# Autodesk Inventor assembly: 조립품2
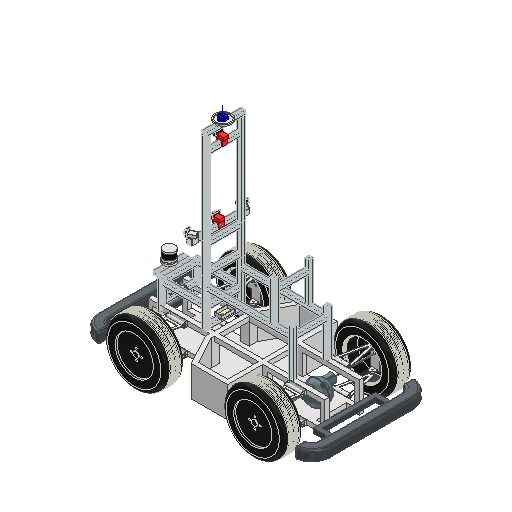
[picture p0: Inventor's stored thumbnail of the model, 512x512]
Saved by Autodesk Inventor 2025.2 (Build 292293000, 293)
## iProperties
Created: 2025-01-26
Part Number: 조립품2
Document SubType Name: Assembly
Designer: jbhma
Author: jbhma
## Documents named in this file (29)
- C:\Users\jbhma\OneDrive\Desktop\2025_ACCA\25_Car\Car1.iam
- C:\Users\jbhma\OneDrive\Desktop\2025_ACCA\2024 ERP42\body.ipt
- C:\Users\jbhma\OneDrive\Desktop\2025_ACCA\2024 ERP42\body_braket.ipt
- C:\Users\jbhma\OneDrive\Desktop\2025_ACCA\2024 ERP42\프로파일\40.5.ipt
- C:\Users\jbhma\OneDrive\Desktop\2025_ACCA\2024 ERP42\프로파일\71.ipt
- C:\Users\jbhma\OneDrive\Desktop\2025_ACCA\2024 ERP42\프로파일\34.ipt
- C:\Users\jbhma\OneDrive\Desktop\2025_ACCA\2024 ERP42\프로파일\26.ipt
- C:\Users\jbhma\OneDrive\Desktop\2025_ACCA\2024 ERP42\프로파일\79.ipt
- C:\Users\jbhma\OneDrive\Desktop\2025_ACCA\2024 ERP42\bumper.ipt
- C:\Users\jbhma\OneDrive\Desktop\2025_ACCA\2024 ERP42\link.ipt
- C:\Users\jbhma\OneDrive\Desktop\2025_ACCA\2024 ERP42\wheel_bolt.ipt
- C:\Users\jbhma\OneDrive\Desktop\2025_ACCA\2024 ERP42\wheel_braket_13.ipt
- C:\Users\jbhma\OneDrive\Desktop\2025_ACCA\2024 ERP42\wheel_braket_24.ipt
- C:\Users\jbhma\OneDrive\Desktop\2025_ACCA\2024 ERP42\wheel.ipt
- C:\Users\jbhma\OneDrive\Desktop\2025_ACCA\2024 ERP42\base_link.ipt
- base_link.ipt
- C:\Users\jbhma\OneDrive\Desktop\2025_ACCA\2024 ERP42\프로파일\50.ipt
- C:\Users\jbhma\OneDrive\Desktop\2025_ACCA\2024 ERP42\camera_case_front.ipt
- C:\Users\jbhma\OneDrive\Desktop\2025_ACCA\2024 ERP42\camera_case_left.ipt
- C:\Users\jbhma\OneDrive\Desktop\2025_ACCA\2024 ERP42\camera_case_right.ipt
- C:\Users\jbhma\OneDrive\Desktop\2025_ACCA\2024 ERP42\camera.ipt
- C:\Users\jbhma\OneDrive\Desktop\2025_ACCA\2024 ERP42\lidar_case.ipt
- C:\Users\jbhma\OneDrive\Desktop\2025_ACCA\2024 ERP42\imu_case_new.ipt
- C:\Users\jbhma\OneDrive\Desktop\2025_ACCA\2024 ERP42\gps_case.ipt
- C:\Users\jbhma\OneDrive\Desktop\2025_ACCA\2024 ERP42\UBLOX_ANN-MB-00_GNSS_ANTENNA.ipt
- C:\Users\jbhma\OneDrive\Desktop\2025_ACCA\2024 ERP42\lidar.ipt
- C:\Users\jbhma\OneDrive\Desktop\2025_ACCA\2024 ERP42\MTi 600-series STEP files\MTi-600 DEV assembly.iam
- C:\Users\jbhma\OneDrive\Desktop\2025_ACCA\2024 ERP42\MTi 600-series STEP files\MTi 1-s DK GNSS.iam
- C:\Users\jbhma\OneDrive\Desktop\2025_ACCA\2024 ERP42\gps_case_2.ipt
## Components (81 placed, 27 different names)
1. body:1 — 메이트:113, 메이트:114, 메이트:115, 메이트:116, 메이트:117, 메이트:118, 메이트:119, 메이트:120, 메이트:124, 메이트:125, 메이트:126, 메이트:127, 메이트:128, 메이트:131, 메이트:137, 메이트:139, 메이트:191, 메이트:192, 메이트:193, 메이트:194, 메이트:195, 메이트:196, 메이트:197, 메이트:198, 메이트:199, 메이트:200, 메이트:201, 메이트:202, 메이트:203, 메이트:204, 메이트:205, 메이트:206
2. body_braket:9 — 메이트:113, 메이트:114, 메이트:212
3. body_braket:10 — 메이트:115, 메이트:116, 메이트:211
4. body_braket:11 — 메이트:117, 메이트:118, 메이트:213
5. body_braket:12 — 메이트:119, 메이트:120, 메이트:214
6. body_braket:13 — 메이트:191, 메이트:195, 메이트:199, 메이트:215
7. body_braket:14 — 메이트:193, 메이트:197, 메이트:202, 메이트:217
8. body_braket:15 — 메이트:194, 메이트:198, 메이트:201, 메이트:218
9. body_braket:16 — 메이트:192, 메이트:196, 메이트:200, 메이트:216
10. bumper:1 — 메이트:203, 메이트:204
11. bumper:2 — 메이트:205, 메이트:206
12. 40.5:12 — 메이트:126, 메이트:127, 메이트:130, 메이트:257
13. 40.5:13 — 메이트:124, 메이트:125, 메이트:129
14. 71:1 — 메이트:128, 메이트:129, 메이트:132, 메이트:133, 메이트:138
15. 71:2 — 메이트:130, 메이트:131, 메이트:134, 메이트:135, 메이트:136, 메이트:256
16. 34:1 — 메이트:134, 메이트:135, 메이트:189
17. 34:2 — 메이트:132, 메이트:133, 메이트:190
18. 40.5:15 — 메이트:136, 메이트:137, 메이트:143, 메이트:144, 메이트:145, 메이트:293
19. 40.5:16 — 메이트:138, 메이트:139, 메이트:140, 메이트:141, 메이트:142, 메이트:168, 메이트:180, 메이트:287, 메이트:288
20. 26:1 — 메이트:140, 메이트:141, 메이트:142, 메이트:149, 메이트:150, 메이트:175, 메이트:176, 메이트:178
21. 26:2 — 메이트:143, 메이트:144, 메이트:145, 메이트:151, 메이트:152, 메이트:177
22. 79:1 — 메이트:151, 메이트:152, 메이트:261
23. 79:2 — 메이트:149, 메이트:150, 메이트:153, 메이트:154, 메이트:262, 각도:3
24. 34:3 — 메이트:153, 메이트:154, 메이트:259
25. 34:6 — 메이트:168, 메이트:172, 각도:1, 메이트:179
26. 34:7 — 메이트:296
27. 26:3 — 메이트:172, 각도:1, 메이트:295, 메이트:297
28. 26:5 — 메이트:175, 메이트:176
29. 26:6 — 메이트:177, 메이트:178, 메이트:301
30. 26:7 — 메이트:179, 메이트:180
31. 26:8 — 메이트:258, 메이트:261, 메이트:262
32. 26:10 — 메이트:189, 메이트:190
33. link:5 — 메이트:211, 메이트:226
34. link:6 — 메이트:212, 메이트:224
35. link:7 — 메이트:214, 메이트:227
36. link:8 — 메이트:213, 메이트:225
37. link:12 — 메이트:215, 메이트:219
38. link:13 — 메이트:217, 메이트:223
39. link:14 — 메이트:216, 메이트:220
40. link:15 — 메이트:218, 메이트:222
41. wheel_bolt:1 — 메이트:219, 메이트:221
42. wheel_braket_13:1 — 메이트:221, 메이트:236, 메이트:237
43. wheel_braket_24:1 — 메이트:229, 메이트:235, 메이트:238
44. wheel_bolt:2 — 메이트:220
45. wheel_bolt:3 — 메이트:222, 메이트:230
46. wheel_bolt:4 — 메이트:223
47. wheel_bolt:5 — 메이트:224, 메이트:228
48. wheel_bolt:6 — 메이트:225, 메이트:229
49. wheel_bolt:7 — 메이트:226
50. wheel_bolt:8 — 메이트:227
51. wheel_braket_13:2 — 메이트:228, 메이트:232
52. wheel:1 — 메이트:232
53. wheel:2 — 메이트:238
54. wheel_braket_24:2 — 메이트:230, 메이트:234
55. wheel:3 — 메이트:237
56. wheel:4 — 메이트:234
57. base_link:1 — 메이트:235, 메이트:236
58. 26:12 — 메이트:256, 메이트:257
59. gps_case:1 — 메이트:259, 각도:3
60. camera_case_front:2 — 메이트:258, 메이트:278
61. UBLOX_ANN-MB-00_GNSS_ANTENNA:1
62. camera:4 — 메이트:278
63. 26:13 — 메이트:290
64. gps_case_2:1 — 메이트:293, 메이트:294, 강체:1
65. MTi 1-s DK GNSS:1 [sub-assembly] — 강체:1
66. 26:14 — 메이트:287, 메이트:288, 메이트:294
67. MTi-600 DEV assembly:1 [sub-assembly] — 메이트:291, 메이트:292
68. imu_case_new:1 — 메이트:290, 메이트:291, 메이트:292
69. 26:15 — 메이트:295, 메이트:298
70. 26:16 — 메이트:296
71. 26:17 — 메이트:297, 메이트:298, 메이트:299, 메이트:300
72. 26:18 — 메이트:299, 메이트:300, 강체:2
73. lidar_case:1 — 강체:2, 회전:1
74. lidar:1 — 회전:1
75. camera:5 — 메이트:306
76. 50:1 — 메이트:301, 메이트:302, 메이트:303, 메이트:304, 메이트:305
77. camera_case_left:1 — 메이트:302, 메이트:306
78. camera_case_front:3 — 메이트:305, 메이트:307
79. camera:6 — 메이트:307
80. camera:7 — 메이트:308
81. camera_case_right:1 — 메이트:303, 메이트:304, 메이트:308
## Relationships (121: Mate 116, Angle 2, WeldJoint 2, RevoluteJoint 1)
- 메이트:113 [Mate] (195 mm): body:1 ↔ body_braket:9
- 메이트:114 [Mate]: body:1 ↔ body_braket:9
- 메이트:115 [Mate] (195 mm): body:1 ↔ body_braket:10
- 메이트:116 [Mate]: body:1 ↔ body_braket:10
- 메이트:117 [Mate] (155 mm): body:1 ↔ body_braket:11
- 메이트:118 [Mate]: body:1 ↔ body_braket:11
- 메이트:119 [Mate] (155 mm): body:1 ↔ body_braket:12
- 메이트:120 [Mate]: body:1 ↔ body_braket:12
- 메이트:124 [Mate]: body:1 ↔ 40.5:13
- 메이트:125 [Mate] (275 mm): body:1 ↔ 40.5:13
- 메이트:126 [Mate]: body:1 ↔ 40.5:12
- 메이트:127 [Mate] (275 mm): body:1 ↔ 40.5:12
- 메이트:128 [Mate] (300 mm): body:1 ↔ 71:1
- 메이트:129 [Mate]: 40.5:13 ↔ 71:1
- 메이트:130 [Mate]: 40.5:12 ↔ 71:2
- 메이트:131 [Mate] (300 mm): body:1 ↔ 71:2
- 메이트:132 [Mate]: 71:1 ↔ 34:2
- 메이트:133 [Mate] (120 mm): 71:1 ↔ 34:2
- 메이트:134 [Mate]: 71:2 ↔ 34:1
- 메이트:135 [Mate] (120 mm): 71:2 ↔ 34:1
- 메이트:136 [Mate]: 71:2 ↔ 40.5:15
- 메이트:137 [Mate]: body:1 ↔ 40.5:15
- 메이트:138 [Mate]: 71:1 ↔ 40.5:16
- 메이트:139 [Mate]: body:1 ↔ 40.5:16
- 메이트:140 [Mate]: 40.5:16 ↔ 26:1
- 메이트:141 [Mate]: 40.5:16 ↔ 26:1
- 메이트:142 [Mate]: 40.5:16 ↔ 26:1
- 메이트:143 [Mate]: 40.5:15 ↔ 26:2
- 메이트:144 [Mate]: 40.5:15 ↔ 26:2
- 메이트:145 [Mate]: 40.5:15 ↔ 26:2
- 메이트:149 [Mate]: 26:1 ↔ 79:2
- 메이트:150 [Mate]: 26:1 ↔ 79:2
- 메이트:151 [Mate]: 26:2 ↔ 79:1
- 메이트:152 [Mate]: 26:2 ↔ 79:1
- 메이트:153 [Mate]: 79:2 ↔ 34:3
- 메이트:154 [Mate]: 79:2 ↔ 34:3
- 메이트:168 [Mate]: 40.5:16 ↔ 34:6
- 메이트:172 [Mate]: 34:6 ↔ 26:3
- 각도:1 [Angle] (90 deg): 34:6 ↔ 26:3
- 메이트:175 [Mate]: 26:1 ↔ 26:5
- 메이트:176 [Mate]: 26:1 ↔ 26:5
- 메이트:177 [Mate]: 26:2 ↔ 26:6
- 메이트:178 [Mate]: 26:1 ↔ 26:6
- 메이트:179 [Mate]: 34:6 ↔ 26:7
- 메이트:180 [Mate]: 40.5:16 ↔ 26:7
- 메이트:189 [Mate]: 34:1 ↔ 26:10
- 메이트:190 [Mate]: 34:2 ↔ 26:10
- 메이트:191 [Mate]: body:1 ↔ body_braket:13
- 메이트:192 [Mate]: body:1 ↔ body_braket:16
- 메이트:193 [Mate]: body:1 ↔ body_braket:14
- 메이트:194 [Mate]: body:1 ↔ body_braket:15
- 메이트:195 [Mate]: body:1 ↔ body_braket:13
- 메이트:196 [Mate]: body:1 ↔ body_braket:16
- 메이트:197 [Mate]: body:1 ↔ body_braket:14
- 메이트:198 [Mate]: body:1 ↔ body_braket:15
- 메이트:199 [Mate] (155 mm): body:1 ↔ body_braket:13
- 메이트:200 [Mate] (155 mm): body:1 ↔ body_braket:16
- 메이트:201 [Mate] (195 mm): body:1 ↔ body_braket:15
- 메이트:202 [Mate] (195 mm): body:1 ↔ body_braket:14
- 메이트:203 [Mate]: body:1 ↔ bumper:1
- 메이트:204 [Mate] (100 mm): body:1 ↔ bumper:1
- 메이트:205 [Mate]: body:1 ↔ bumper:2
- 메이트:206 [Mate] (100 mm): body:1 ↔ bumper:2
- 메이트:211 [Mate]: body_braket:10 ↔ link:5
- 메이트:212 [Mate]: body_braket:9 ↔ link:6
- 메이트:213 [Mate]: body_braket:11 ↔ link:8
- 메이트:214 [Mate]: body_braket:12 ↔ link:7
- 메이트:215 [Mate]: body_braket:13 ↔ link:12
- 메이트:216 [Mate]: body_braket:16 ↔ link:14
- 메이트:217 [Mate]: body_braket:14 ↔ link:13
- 메이트:218 [Mate]: body_braket:15 ↔ link:15
- 메이트:219 [Mate]: link:12 ↔ wheel_bolt:1
- 메이트:220 [Mate]: link:14 ↔ wheel_bolt:2
- 메이트:221 [Mate]: wheel_bolt:1 ↔ wheel_braket_13:1
- 메이트:222 [Mate]: link:15 ↔ wheel_bolt:3
- 메이트:223 [Mate]: link:13 ↔ wheel_bolt:4
- 메이트:224 [Mate]: link:6 ↔ wheel_bolt:5
- 메이트:225 [Mate]: link:8 ↔ wheel_bolt:6
- 메이트:226 [Mate]: link:5 ↔ wheel_bolt:7
- 메이트:227 [Mate]: link:7 ↔ wheel_bolt:8
- 메이트:228 [Mate]: wheel_bolt:5 ↔ wheel_braket_13:2
- 메이트:229 [Mate]: wheel_braket_24:1 ↔ wheel_bolt:6
- 메이트:230 [Mate]: wheel_bolt:3 ↔ wheel_braket_24:2
- 메이트:232 [Mate]: wheel_braket_13:2 ↔ wheel:1
- 메이트:234 [Mate]: wheel_braket_24:2 ↔ wheel:4
- 메이트:235 [Mate]: wheel_braket_24:1 ↔ base_link:1
- 메이트:236 [Mate]: wheel_braket_13:1 ↔ base_link:1
- 메이트:237 [Mate]: wheel_braket_13:1 ↔ wheel:3
- 메이트:238 [Mate]: wheel_braket_24:1 ↔ wheel:2
- 메이트:256 [Mate]: 71:2 ↔ 26:12
- 메이트:257 [Mate]: 40.5:12 ↔ 26:12
- 메이트:258 [Mate]: 26:8 ↔ camera_case_front:2
- 메이트:259 [Mate]: 34:3 ↔ gps_case:1
- 메이트:261 [Mate]: 79:1 ↔ 26:8
- 메이트:262 [Mate]: 79:2 ↔ 26:8
- 각도:3 [Angle] (90 deg): 79:2 ↔ gps_case:1
- 메이트:278 [Mate]: camera_case_front:2 ↔ camera:4
- 메이트:287 [Mate]: 40.5:16 ↔ 26:14
- 메이트:288 [Mate]: 40.5:16 ↔ 26:14
- 메이트:290 [Mate]: 26:13 ↔ imu_case_new:1
- 메이트:291 [Mate]: MTi-600 DEV assembly:1 ↔ imu_case_new:1
- 메이트:292 [Mate]: MTi-600 DEV assembly:1 ↔ imu_case_new:1
- 메이트:293 [Mate] (72.5 mm): 40.5:15 ↔ gps_case_2:1
- 메이트:294 [Mate]: gps_case_2:1 ↔ 26:14
- 강체:1 [WeldJoint]: gps_case_2:1 ↔ MTi 1-s DK GNSS:1
- 메이트:295 [Mate]: 26:3 ↔ 26:15
- 메이트:296 [Mate]: 34:7 ↔ 26:16
- 메이트:297 [Mate]: 26:3 ↔ 26:17
- 메이트:298 [Mate]: 26:15 ↔ 26:17
- 메이트:299 [Mate]: 26:17 ↔ 26:18
- 메이트:300 [Mate]: 26:17 ↔ 26:18
- 강체:2 [WeldJoint]: 26:18 ↔ lidar_case:1
- 회전:1 [RevoluteJoint]: lidar_case:1 ↔ lidar:1
- 메이트:301 [Mate]: 26:6 ↔ 50:1
- 메이트:302 [Mate]: 50:1 ↔ camera_case_left:1
- 메이트:303 [Mate]: 50:1 ↔ camera_case_right:1
- 메이트:304 [Mate]: 50:1 ↔ camera_case_right:1
- 메이트:305 [Mate]: 50:1 ↔ camera_case_front:3
- 메이트:306 [Mate]: camera:5 ↔ camera_case_left:1
- 메이트:307 [Mate]: camera_case_front:3 ↔ camera:6
- 메이트:308 [Mate]: camera:7 ↔ camera_case_right:1
